# Autodesk Inventor assembly: chwytak_podstawa
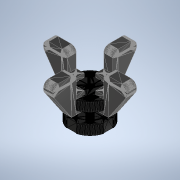
[picture p0: Inventor's stored thumbnail of the model, 180x180]
Saved by Autodesk Inventor 2022.3 (Build 263350000, 350)
## iProperties
Created: 2023-06-03
Part Number: chwytak_podstawa
Document SubType Name: Assembly
Designer: komputer
Author: komputer
## Documents named in this file (5)
- C:\Users\komputer\Documents\Inventor\chwytak\chwytak_podstawa.iam
- C:\Users\komputer\Documents\Inventor\chwytak\GripperBaseCircularLower.ipt
- C:\Users\komputer\Documents\Inventor\chwytak\GripperBaseCircularUpper.ipt
- C:\Users\komputer\Documents\Inventor\chwytak\CircularStandOff.ipt
- C:\Users\komputer\Documents\Inventor\chwytak\ClawShoulder.ipt
## Components (10 placed, 4 different names)
1. GripperBaseCircularLower:1 — Mate:1, Mate:2, Mate:3, Mate:4, Mate:5, Mate:6, Mate:7, Mate:23
2. GripperBaseCircularUpper:1 — Mate:8, Mate:11, Mate:13, Mate:14, Mate:15, Mate:16, Mate:18, Mate:20, Mate:22, Mate:24
3. CircularStandOff:1 — Mate:1, Mate:23
4. ClawShoulder:1 — Mate:16, Mate:22, Flush:1
5. CircularStandOff:2 — Mate:4, Mate:7, Mate:8
6. CircularStandOff:3 — Mate:2, Mate:5
7. CircularStandOff:4 — Mate:3, Mate:6, Mate:24
8. ClawShoulder:2 — Mate:11, Mate:13, Flush:2
9. ClawShoulder:3 — Mate:15, Mate:18, Flush:1
10. ClawShoulder:4 — Mate:14, Mate:20, Flush:2
## Relationships (20: Mate 18, Flush 2)
- Mate:1: GripperBaseCircularLower:1 ↔ CircularStandOff:1
- Mate:2: GripperBaseCircularLower:1 ↔ CircularStandOff:3
- Mate:3: GripperBaseCircularLower:1 ↔ CircularStandOff:4
- Mate:4: GripperBaseCircularLower:1 ↔ CircularStandOff:2
- Mate:5: GripperBaseCircularLower:1 ↔ CircularStandOff:3
- Mate:6: GripperBaseCircularLower:1 ↔ CircularStandOff:4
- Mate:7: GripperBaseCircularLower:1 ↔ CircularStandOff:2
- Mate:8: GripperBaseCircularUpper:1 ↔ CircularStandOff:2
- Mate:11: GripperBaseCircularUpper:1 ↔ ClawShoulder:2
- Mate:13: GripperBaseCircularUpper:1 ↔ ClawShoulder:2
- Mate:14: GripperBaseCircularUpper:1 ↔ ClawShoulder:4
- Mate:15: GripperBaseCircularUpper:1 ↔ ClawShoulder:3
- Mate:16: GripperBaseCircularUpper:1 ↔ ClawShoulder:1
- Mate:18: GripperBaseCircularUpper:1 ↔ ClawShoulder:3
- Mate:20: GripperBaseCircularUpper:1 ↔ ClawShoulder:4
- Mate:22: GripperBaseCircularUpper:1 ↔ ClawShoulder:1
- Mate:23: GripperBaseCircularLower:1 ↔ CircularStandOff:1
- Flush:1: ClawShoulder:1 ↔ ClawShoulder:3
- Flush:2: ClawShoulder:2 ↔ ClawShoulder:4
- Mate:24: GripperBaseCircularUpper:1 ↔ CircularStandOff:4
